# Autodesk Inventor assembly: Leg_joint_roll_yaw
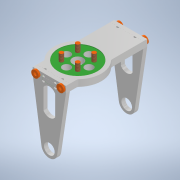
[picture p0: Inventor's stored thumbnail of the model, 180x180]
Saved by Autodesk Inventor 2020 (Build 240168000, 168)
## iProperties
Created: 2022-06-14
Part Number: Leg_joint_roll_yaw
Document SubType Name: Assembly
Designer: Masato Kubotera
Author: Masato Kubotera
## Documents named in this file (5)
- C:\Users\MasatoKubotera\Documents\Inventor\SUSTAINA-OP\LowerBody\Leg_joint\Leg_joint_roll_yaw.iam
- C:\Users\MasatoKubotera\Documents\Inventor\SUSTAINA-OP\LowerBody\Leg_joint\Leg_joint_slider_frame.ipt
- C:\Users\MasatoKubotera\Documents\Inventor\SUSTAINA-OP\LowerBody\Leg_joint\Leg_joint_yaw_frame.ipt
- C:\Users\MasatoKubotera\Documents\Inventor\SUSTAINA-OP\ReadyMade\Screw\M3-10.ipt
- C:\Users\MasatoKubotera\Documents\Inventor\SUSTAINA-OP\ReadyMade\Screw\M3-6.ipt
## Components (11 placed, 4 different names)
1. Leg_joint_yaw_frame:1 — メイト:2, フラッシュ:2, フラッシュ:3, 挿入:1, 挿入:2, 挿入:3, 挿入:4, 挿入:5, 挿入:6, 挿入:7, 挿入:8
2. Leg_joint_slider_frame:1 — 挿入:1, 挿入:2, 挿入:9, 挿入:10
3. Leg_joint_slider_frame:2 — 挿入:3, 挿入:4, 挿入:11, 挿入:12
4. M3-10:1 — 挿入:5
5. M3-10:2 — 挿入:6
6. M3-10:3 — 挿入:7
7. M3-10:4 — 挿入:8
8. M3-6:1 — 挿入:9
9. M3-6:2 — 挿入:10
10. M3-6:3 — 挿入:11
11. M3-6:4 — 挿入:12
## Relationships (15: Insert 12, Flush 2, Mate 1)
- メイト:2 [Mate]: Leg_joint_yaw_frame:1
- フラッシュ:2 [Flush]: Leg_joint_yaw_frame:1
- フラッシュ:3 [Flush]: Leg_joint_yaw_frame:1
- 挿入:1 [Insert]: Leg_joint_yaw_frame:1 ↔ Leg_joint_slider_frame:1
- 挿入:2 [Insert]: Leg_joint_yaw_frame:1 ↔ Leg_joint_slider_frame:1
- 挿入:3 [Insert]: Leg_joint_yaw_frame:1 ↔ Leg_joint_slider_frame:2
- 挿入:4 [Insert]: Leg_joint_yaw_frame:1 ↔ Leg_joint_slider_frame:2
- 挿入:5 [Insert]: Leg_joint_yaw_frame:1 ↔ M3-10:1
- 挿入:6 [Insert]: Leg_joint_yaw_frame:1 ↔ M3-10:2
- 挿入:7 [Insert]: Leg_joint_yaw_frame:1 ↔ M3-10:3
- 挿入:8 [Insert]: Leg_joint_yaw_frame:1 ↔ M3-10:4
- 挿入:9 [Insert]: Leg_joint_slider_frame:1 ↔ M3-6:1
- 挿入:10 [Insert]: Leg_joint_slider_frame:1 ↔ M3-6:2
- 挿入:11 [Insert]: Leg_joint_slider_frame:2 ↔ M3-6:3
- 挿入:12 [Insert]: Leg_joint_slider_frame:2 ↔ M3-6:4
